# Autodesk Inventor assembly: Assembly3
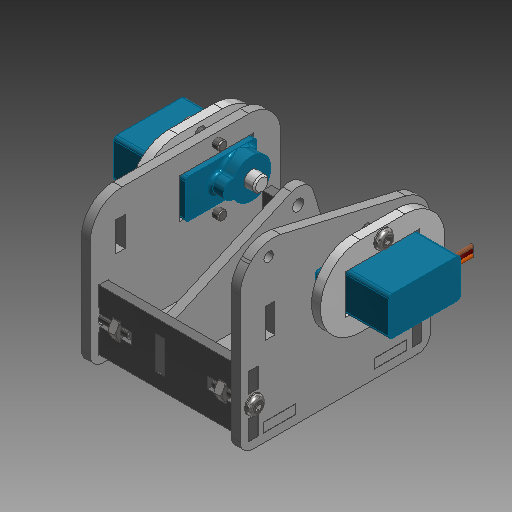
[picture p0: Inventor's stored thumbnail of the model, 512x512]
Saved by Autodesk Inventor 2019.2 (Build 232265000, 265)
## iProperties
Part Number: Assembly3
Document SubType Name: Assembly
Designer: richard.girt
Mass: 55.9502 g
Surface Area: 353.65 cm^2
Volume: 44.9491 cm^3
Density: 1.24475 g/cm^3
Author: richard.girt
## Documents named in this file (15)
- C:\Users\richard.girt\Desktop\2 Axis robotic arm\Assembly3.iam
- C:\Users\richard.girt\Desktop\2 Axis robotic arm\Part1.ipt
- C:\Users\richard.girt\Desktop\2 Axis robotic arm\Part9.ipt
- C:\Users\richard.girt\Desktop\2 Axis robotic arm\SG90.ipt
- C:\Users\richard.girt\Desktop\2 Axis robotic arm\Part11.ipt
- C:\Users\richard.girt\Desktop\2 Axis robotic arm\Part13.ipt
- C:\Users\richard.girt\Desktop\2 Axis robotic arm\Part12.ipt
- C:\Users\richard.girt\Desktop\2 Axis robotic arm\SG90Horn2.ipt
- C:\Users\richard.girt\Desktop\2 Axis robotic arm\ANSI B18.6.5M - M2.5x0.45 x 4(38).ipt
- C:\Users\richard.girt\Desktop\2 Axis robotic arm\ANSI B18.6.5M - M2.5x0.45 x 8(38).ipt
- ANSI B18.6.5M - M2.5x0.45 x 8(38).ipt
- C:\Users\richard.girt\Desktop\2 Axis robotic arm\Part15.ipt
- C:\Users\richard.girt\Desktop\2 Axis robotic arm\ANSI B 18.2.4.1 M - M3 x 0.5Style 1.ipt
- C:\Users\richard.girt\Desktop\2 Axis robotic arm\ANSI B18.3.4M - M3 x 0.5 x 12(1).ipt
- C:\Users\richard.girt\Desktop\2 Axis robotic arm\ANSI B18.3.4M - M3 x 0.5 x 8(1).ipt
## Components (26 placed, 13 different names)
1. Part12:1 — Mate:1, Mate:2, Flush:1, Flush:2, Flush:3, Flush:4, Flush:9, Flush:12, Rigid:1, Mate:16, Mate:17, Flush:16
2. SG90:1 — Mate:3, Mate:4, Mate:5, Mate:8
3. Part11:1 — Mate:6, Mate:7, Mate:8, Flush:2, Flush:3, Flush:4, Flush:7, Flush:8, Flush:10, Flush:11, Flush:14, Flush:15, Rigid:21, Rigid:22, Rigid:23, Rigid:24
4. Part1:2 — Mate:3, Mate:4, Mate:5, Mate:6, Mate:7, Rigid:13, Rigid:16
5. Part13:1 — Flush:7, Flush:8, Flush:9, Flush:13
6. Part13:2 — Flush:10, Flush:11, Flush:12
7. SG90:2 — Mate:13
8. Part1:3 — Mate:14, Mate:15, Rigid:14, Rigid:15
9. Part9:1 — Flush:13, Flush:14, Flush:15, Mate:13, Mate:14, Mate:15, Rigid:17, Rigid:18, Rigid:19, Rigid:20
10. SG90Horn2:1 — Rigid:1, Rigid:2, Rigid:3, Rigid:4
11. ANSI B18.6.5M - M2.5x0.45 x 4(38):1 — Rigid:2
12. ANSI B18.6.5M - M2.5x0.45 x 8(38):1 — Rigid:3
13. ANSI B18.6.5M - M2.5x0.45 x 8(38):2 — Rigid:4
14. Part15:1 — Mate:16, Mate:17, Flush:16
15. ANSI B 18.2.4.1 M - M3 x 0.5Style 1:1 — Rigid:20
16. ANSI B 18.2.4.1 M - M3 x 0.5Style 1:2 — Rigid:24
17. ANSI B 18.2.4.1 M - M3 x 0.5Style 1:3 — Rigid:21
18. ANSI B 18.2.4.1 M - M3 x 0.5Style 1:4 — Rigid:19
19. ANSI B18.3.4M - M3 x 0.5 x 12(1):1 — Rigid:23
20. ANSI B18.3.4M - M3 x 0.5 x 12(1):2 — Rigid:22
21. ANSI B18.3.4M - M3 x 0.5 x 12(1):3 — Rigid:17
22. ANSI B18.3.4M - M3 x 0.5 x 12(1):4 — Rigid:18
23. ANSI B18.3.4M - M3 x 0.5 x 8(1):1 — Rigid:13
24. ANSI B18.3.4M - M3 x 0.5 x 8(1):2 — Rigid:16
25. ANSI B18.3.4M - M3 x 0.5 x 8(1):3 — Rigid:14
26. ANSI B18.3.4M - M3 x 0.5 x 8(1):4 — Rigid:15
## Relationships (46: Mate 16, WeldJoint 16, Flush 14)
- Mate:1: Part12:1
- Mate:2: Part12:1
- Flush:1: Part12:1
- Mate:3: SG90:1 ↔ Part1:2
- Mate:4: SG90:1 ↔ Part1:2
- Mate:5: SG90:1 ↔ Part1:2
- Mate:6: Part11:1 ↔ Part1:2
- Mate:7: Part11:1 ↔ Part1:2
- Mate:8: SG90:1 ↔ Part11:1
- Flush:2: Part12:1 ↔ Part11:1
- Flush:3: Part12:1 ↔ Part11:1
- Flush:4 (2.8 mm): Part12:1 ↔ Part11:1
- Flush:7: Part11:1 ↔ Part13:1
- Flush:8 (2.8 mm): Part11:1 ↔ Part13:1
- Flush:9: Part12:1 ↔ Part13:1
- Flush:10: Part11:1 ↔ Part13:2
- Flush:11 (2.8 mm): Part11:1 ↔ Part13:2
- Flush:12: Part12:1 ↔ Part13:2
- [Mate]: SG90:2 ↔ Part1:3
- [Mate]: SG90:2 ↔ Part1:3
- [Mate]: SG90:2 ↔ Part1:3
- Flush:13: Part13:1 ↔ Part9:1
- Flush:14: Part11:1 ↔ Part9:1
- Flush:15: Part11:1 ↔ Part9:1
- Mate:13: SG90:2 ↔ Part9:1
- Mate:14: Part1:3 ↔ Part9:1
- Mate:15: Part1:3 ↔ Part9:1
- Rigid:1 [WeldJoint]: Part12:1 ↔ SG90Horn2:1
- Rigid:2 [WeldJoint]: SG90Horn2:1 ↔ ANSI B18.6.5M - M2.5x0.45 x 4(38):1
- Rigid:3 [WeldJoint] (2.8 mm): SG90Horn2:1 ↔ ANSI B18.6.5M - M2.5x0.45 x 8(38):1
- Rigid:4 [WeldJoint] (2.8 mm): SG90Horn2:1 ↔ ANSI B18.6.5M - M2.5x0.45 x 8(38):2
- Mate:16: Part12:1 ↔ Part15:1
- Mate:17: Part12:1 ↔ Part15:1
- Flush:16 (20.5 mm): Part12:1 ↔ Part15:1
- Rigid:13 [WeldJoint]: Part1:2 ↔ ANSI B18.3.4M - M3 x 0.5 x 8(1):1
- Rigid:14 [WeldJoint]: Part1:3 ↔ ANSI B18.3.4M - M3 x 0.5 x 8(1):3
- Rigid:15 [WeldJoint]: Part1:3 ↔ ANSI B18.3.4M - M3 x 0.5 x 8(1):4
- Rigid:16 [WeldJoint]: Part1:2 ↔ ANSI B18.3.4M - M3 x 0.5 x 8(1):2
- Rigid:17 [WeldJoint]: Part9:1 ↔ ANSI B18.3.4M - M3 x 0.5 x 12(1):3
- Rigid:18 [WeldJoint]: Part9:1 ↔ ANSI B18.3.4M - M3 x 0.5 x 12(1):4
- Rigid:19 [WeldJoint] (-4.3 mm): Part9:1 ↔ ANSI B 18.2.4.1 M - M3 x 0.5Style 1:4
- Rigid:20 [WeldJoint] (-4.3 mm): Part9:1 ↔ ANSI B 18.2.4.1 M - M3 x 0.5Style 1:1
- Rigid:21 [WeldJoint] (-4.3 mm): Part11:1 ↔ ANSI B 18.2.4.1 M - M3 x 0.5Style 1:3
- Rigid:22 [WeldJoint]: Part11:1 ↔ ANSI B18.3.4M - M3 x 0.5 x 12(1):2
- Rigid:23 [WeldJoint]: Part11:1 ↔ ANSI B18.3.4M - M3 x 0.5 x 12(1):1
- Rigid:24 [WeldJoint] (-4.3 mm): Part11:1 ↔ ANSI B 18.2.4.1 M - M3 x 0.5Style 1:2
## Named parameters: d22_d6 = 0 mm, d23_d3 = 0 mm, d24_d4 = 0 mm
